# Autodesk Inventor assembly: HubWheel-6_5_asm
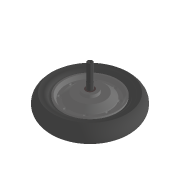
[picture p0: Inventor's stored thumbnail of the model, 180x180]
Saved by Autodesk Inventor 2022 (Build 260153000, 153)
## iProperties
Created: 2025-01-12
Part Number: HubWheel-6_5_asm
Document SubType Name: Assembly
Designer: Home
Author: Home
## Documents named in this file (7)
- D:\YandexDisk\Voltbro\xSets\components\HubWheel-10\HubWheel-10_asm.iam
- D:\YandexDisk\Voltbro\xSets\components\HubWheel-10\stator-assembly.iam
- D:\YandexDisk\Voltbro\xSets\components\HubWheel-10\rotor-housing-assembly.iam
- D:\YandexDisk\Voltbro\xSets\components\HubWheel-10\components\bearings\6003-2rs_17x35x10.ipt
- D:\YandexDisk\Voltbro\xSets\components\HubWheel-10\components\seal-ring-17x25x5.ipt
- D:\YandexDisk\Voltbro\xSets\components\HubWheel-10\rotor-back-lid.ipt
- D:\YandexDisk\Voltbro\xSets\components\HubWheel-10\tyre-10x2_125.ipt
## Components (6 placed, 6 different names)
1. stator-assembly:1 [sub-assembly] — Mate:1, Flush:1, Angle:1, Insert:1
2. rotor-housing-assembly:1 [sub-assembly] — Insert:1, Insert:4, Mate:2, Insert:5
3. 6003-2rs_17x35x10:1 — Insert:3
4. seal-ring-17x25x5:1 — Insert:2
5. rotor-back-lid:1 — Insert:2, Insert:3, Insert:4, Mate:2
6. tyre-10x2_125:1 — Insert:5
## Relationships (9: Insert 5, Mate 2, Flush 1, Angle 1)
- Mate:1: stator-assembly:1
- Flush:1: stator-assembly:1
- Angle:1 (0 deg): stator-assembly:1
- Insert:1: stator-assembly:1 ↔ rotor-housing-assembly:1
- Insert:2: seal-ring-17x25x5:1 ↔ rotor-back-lid:1
- Insert:3: 6003-2rs_17x35x10:1 ↔ rotor-back-lid:1
- Insert:4: rotor-housing-assembly:1 ↔ rotor-back-lid:1
- Mate:2: rotor-housing-assembly:1 ↔ rotor-back-lid:1
- Insert:5: rotor-housing-assembly:1 ↔ tyre-10x2_125:1
